# Autodesk Inventor assembly: Frame and Wheels
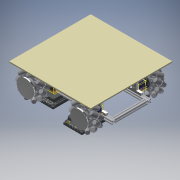
[picture p0: Inventor's stored thumbnail of the model, 180x180]
Saved by Autodesk Inventor 2019 (Build 230136000, 136)
## iProperties
Created: 2019-03-05
Part Number: Frame and Wheels
Document SubType Name: Assembly
Designer: Delta
Mass: 6618.59 g
Surface Area: 22940.3 cm^2
Volume: 3791.34 cm^3
Density: 1.74571 g/cm^3
Author: Delta
## Documents named in this file (7)
- C:\Robotics\2019-20_CAD\offseason\drive train\Frame and Wheels.iam
- C:\Robotics\2019-20_CAD\offseason\drive train\Wheel Sub-Assembly.iam
- C:\Robotics\2019-20_CAD\offseason\drive train\Motor Block.ipt
- C:\Robotics\COTSParts\Bosch Extrusion\Bosch 20x20 17.5 in.ipt
- C:\Robotics\COTSParts\Bosch Extrusion\Bosch 20x20 6.75 in.ipt
- C:\Robotics\2019-20_CAD\offseason\drive train\Top Plate.ipt
- C:\Robotics\COTSParts\Rev\REV-31-1153RevHub.ipt
## Components (16 placed, 6 different names)
1. Wheel Sub-Assembly:1 [sub-assembly] — Insert:2, Angle:2
2. Wheel Sub-Assembly:2 [sub-assembly] — Insert:4, Angle:4
3. Wheel Sub-Assembly:3 [sub-assembly] — Insert:1, Angle:1
4. Wheel Sub-Assembly:4 [sub-assembly] — Insert:3, Angle:3
5. Motor Block:1 — Insert:1, Mate:1, Flush:1, Mate:2, Angle:1
6. Motor Block:2 — Insert:3, Mate:5, Flush:3, Mate:6, Angle:3, Mate:14, Flush:12
7. Motor Block:3 — Insert:2, Mate:3, Flush:2, Mate:4, Angle:2
8. Motor Block:4 — Mate:7, Flush:4, Mate:8, Insert:4, Angle:4
9. Bosch 20x20 17.5 in:1 — Mate:1, Flush:1, Mate:2, Mate:3, Flush:2, Mate:4, Mate:9, Flush:7, Flush:8, Flush:9, Mate:11, Mate:12, Symmetry:1
10. Bosch 20x20 17.5 in:2 — Mate:5, Flush:3, Mate:6, Mate:7, Flush:4, Mate:8, Flush:5, Flush:6, Mate:10, Flush:10, Flush:11, Symmetry:1
11. Bosch 20x20 6.75 in:1 — Flush:9, Mate:10, Mate:11, Flush:10, Mate:13
12. Bosch 20x20 6.75 in:2 — Flush:5, Flush:6, Mate:9, Flush:7, Flush:8
13. Bosch 20x20 6.75 in:3 — Flush:11, Mate:12, Mate:13
14. Top Plate:1 — Mate:14, Flush:12, Mate:15
15. REV-31-1153RevHub:1
16. REV-31-1153RevHub:2
## Relationships (36: Mate 15, Flush 12, Insert 4, Angle 4, Symmetry 1)
- Insert:1: Wheel Sub-Assembly:3 ↔ Motor Block:1
- Mate:1: Motor Block:1 ↔ Bosch 20x20 17.5 in:1
- Flush:1 (3.65 mm): Motor Block:1 ↔ Bosch 20x20 17.5 in:1
- Mate:2 (-76.2 mm): Motor Block:1 ↔ Bosch 20x20 17.5 in:1
- Insert:2: Wheel Sub-Assembly:1 ↔ Motor Block:3
- Angle:1 (180 deg): Wheel Sub-Assembly:3 ↔ Motor Block:1
- Mate:3: Motor Block:3 ↔ Bosch 20x20 17.5 in:1
- Flush:2 (3.65 mm): Motor Block:3 ↔ Bosch 20x20 17.5 in:1
- Mate:4 (-76.2 mm): Motor Block:3 ↔ Bosch 20x20 17.5 in:1
- Angle:2 (0 deg): Wheel Sub-Assembly:1 ↔ Motor Block:3
- Insert:3: Wheel Sub-Assembly:4 ↔ Motor Block:2
- Mate:5: Motor Block:2 ↔ Bosch 20x20 17.5 in:2
- Flush:3 (-3.65 mm): Motor Block:2 ↔ Bosch 20x20 17.5 in:2
- Mate:6 (-76.2 mm): Motor Block:2 ↔ Bosch 20x20 17.5 in:2
- Angle:3 (0 deg): Wheel Sub-Assembly:4 ↔ Motor Block:2
- Mate:7: Motor Block:4 ↔ Bosch 20x20 17.5 in:2
- Flush:4 (3.65 mm): Motor Block:4 ↔ Bosch 20x20 17.5 in:2
- Mate:8 (-76.2 mm): Motor Block:4 ↔ Bosch 20x20 17.5 in:2
- Insert:4: Wheel Sub-Assembly:2 ↔ Motor Block:4
- Angle:4 (180 deg): Wheel Sub-Assembly:2 ↔ Motor Block:4
- Flush:5: Bosch 20x20 17.5 in:2 ↔ Bosch 20x20 6.75 in:2
- Flush:6: Bosch 20x20 17.5 in:2 ↔ Bosch 20x20 6.75 in:2
- Mate:9: Bosch 20x20 17.5 in:1 ↔ Bosch 20x20 6.75 in:2
- Flush:7: Bosch 20x20 17.5 in:1 ↔ Bosch 20x20 6.75 in:2
- Flush:8: Bosch 20x20 17.5 in:1 ↔ Bosch 20x20 6.75 in:2
- Flush:9: Bosch 20x20 17.5 in:1 ↔ Bosch 20x20 6.75 in:1
- Mate:10: Bosch 20x20 17.5 in:2 ↔ Bosch 20x20 6.75 in:1
- Mate:11: Bosch 20x20 17.5 in:1 ↔ Bosch 20x20 6.75 in:1
- Flush:10: Bosch 20x20 17.5 in:2 ↔ Bosch 20x20 6.75 in:1
- Flush:11: Bosch 20x20 17.5 in:2 ↔ Bosch 20x20 6.75 in:3
- Mate:12: Bosch 20x20 17.5 in:1 ↔ Bosch 20x20 6.75 in:3
- Mate:13 (190.5 mm): Bosch 20x20 6.75 in:1 ↔ Bosch 20x20 6.75 in:3
- Mate:14: Motor Block:2 ↔ Top Plate:1
- Flush:12 (-63.5 mm): Motor Block:2 ↔ Top Plate:1
- Symmetry:1: Bosch 20x20 17.5 in:1 ↔ Bosch 20x20 17.5 in:2
- Mate:15 (-222.25 mm): Top Plate:1
